# Autodesk Inventor assembly: Pendulum_No_Wheels
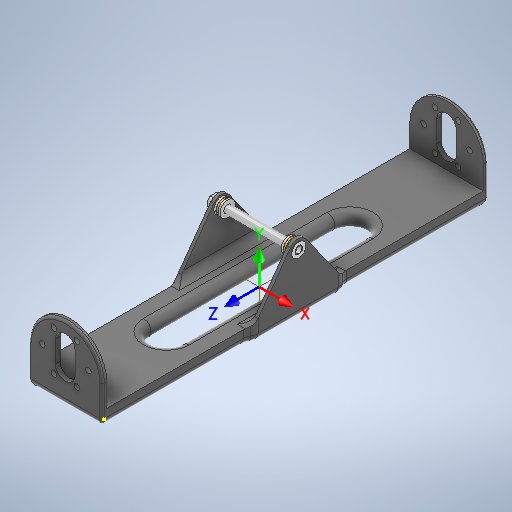
[picture p0: Inventor's stored thumbnail of the model, 512x512]
Saved by Autodesk Inventor 2025.2 (Build 292293000, 293)
## iProperties
Created: 2025-01-23
Part Number: Pendulum_No_Wheels
Document SubType Name: Assembly
Designer: Matt Tidd
Author: Matt Tidd
## Documents named in this file (5)
- C:\Users\mtidd2\Desktop\H2A\CAD\Motors_and_Wheels\Pendulum Suspension\Pendulum_No_Wheels.iam
- C:\Users\mtidd2\Desktop\H2A\CAD\Motors_and_Wheels\Pendulum Suspension\Pendulum Bottom Bracket.ipt
- C:\Users\mtidd2\Desktop\H2A\CAD\Motors_and_Wheels\Pendulum Suspension\Rotation Pin.ipt
- C:\Users\mtidd2\Desktop\H2A\CAD\Motors_and_Wheels\Pendulum Suspension\Rotation Bearing.ipt
- C:\Users\mtidd2\Desktop\H2A\CAD\Motors_and_Wheels\Pendulum Suspension\Rotation End Cap.ipt
## Components (6 placed, 4 different names)
1. Pendulum Bottom Bracket:1 — Flush:3, Mate:1, Mate:2
2. Rotation Bearing:1 — Mate:4
3. Rotation Bearing:2 — Mate:5
4. Rotation End Cap:1 — Mate:2, Mate:5
5. Rotation End Cap:2 — Mate:1, Mate:3, Mate:4
6. Rotation Pin:1 — Mate:3
## Relationships (8: Mate 5, Flush 3)
- [Flush]: Pendulum Bottom Bracket:1
- [Flush]: Pendulum Bottom Bracket:1
- Flush:3: Pendulum Bottom Bracket:1
- Mate:1: Pendulum Bottom Bracket:1 ↔ Rotation End Cap:2
- Mate:2: Pendulum Bottom Bracket:1 ↔ Rotation End Cap:1
- Mate:3: Rotation End Cap:2 ↔ Rotation Pin:1
- Mate:4: Rotation Bearing:1 ↔ Rotation End Cap:2
- Mate:5: Rotation Bearing:2 ↔ Rotation End Cap:1
